# Autodesk Inventor assembly: gun 3_ЗЕРКАЛО1
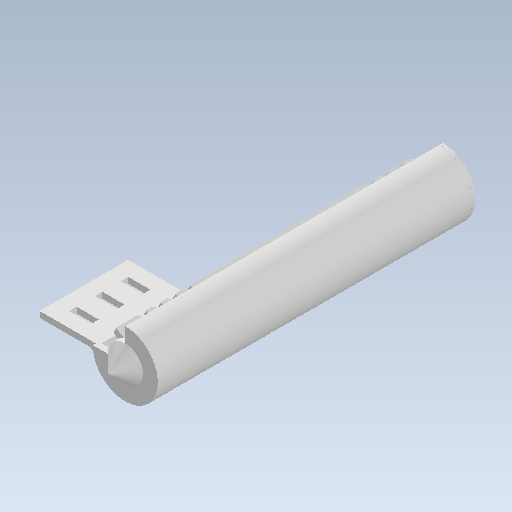
[picture p0: Inventor's stored thumbnail of the model, 512x512]
Saved by Autodesk Inventor 2020.1 (Build 241239000, 239)
## iProperties
Created: 2022-04-02
Part Number: gun 3_ЗЕРКАЛО1
Document SubType Name: Assembly
Designer: User
Author: User
## Documents named in this file (8)
- D:\GitHub\TANK\3D-turret\gun 3_ЗЕРКАЛО1.iam
- D:\GitHub\TANK\3D-turret\barrel_holder_ЗЕРКАЛО1.ipt
- D:\GitHub\TANK\3D-turret\trunk_ЗЕРКАЛО1.ipt
- D:\GitHub\TANK\3D-turret\ось пушки 3_ЗЕРКАЛО1.ipt
- D:\GitHub\TANK\3D-turret\подшипник_ЗЕРКАЛО1.ipt
- D:\GitHub\TANK\3D-turret\кожух пушки_ЗЕРКАЛО1.ipt
- D:\GitHub\TANK\3D-turret\крышка кожуха пушки_ЗЕРКАЛО1.ipt
- D:\GitHub\TANK\3D-turret\крышка кожуха пушки_ЗЕРКАЛО_ЗЕРКАЛО.ipt
## Components (14 placed, 7 different names)
1. barrel_holder_ЗЕРКАЛО1:1 — Жесткий:1, Жесткий:3
2. barrel_holder_ЗЕРКАЛО1:2 — Жесткий:2
3. ось пушки 3_ЗЕРКАЛО1:1 — Жесткий:3, Жесткий:4, Жесткий:5
4. подшипник_ЗЕРКАЛО1:1 — Жесткий:4
5. подшипник_ЗЕРКАЛО1:2 — Совмещение:1, Жесткий:5
6. кожух пушки_ЗЕРКАЛО1:1 — Жесткий:6, Жесткий:7
7. крышка кожуха пушки_ЗЕРКАЛО1:1 — Жесткий:6
8. крышка кожуха пушки_ЗЕРКАЛО_ЗЕРКАЛО:1 — Совмещение:1, Жесткий:7
9. trunk_ЗЕРКАЛО1:1 — Жесткий:1
10. trunk_ЗЕРКАЛО1:2
11. trunk_ЗЕРКАЛО1:3 — Жесткий:2
12. trunk_ЗЕРКАЛО1:4
13. trunk_ЗЕРКАЛО1:5
14. trunk_ЗЕРКАЛО1:6
## Component patterns: (6 elements, first: trunk_ЗЕРКАЛО1:1)
## Relationships (8: WeldJoint 7, Mate 1)
- Совмещение:1 [Mate]: подшипник_ЗЕРКАЛО1:2 ↔ крышка кожуха пушки_ЗЕРКАЛО_ЗЕРКАЛО:1
- Жесткий:1 [WeldJoint]: barrel_holder_ЗЕРКАЛО1:1 ↔ trunk_ЗЕРКАЛО1:1
- Жесткий:3 [WeldJoint]: barrel_holder_ЗЕРКАЛО1:1 ↔ ось пушки 3_ЗЕРКАЛО1:1
- Жесткий:4 [WeldJoint]: ось пушки 3_ЗЕРКАЛО1:1 ↔ подшипник_ЗЕРКАЛО1:1
- Жесткий:5 [WeldJoint]: ось пушки 3_ЗЕРКАЛО1:1 ↔ подшипник_ЗЕРКАЛО1:2
- Жесткий:6 [WeldJoint]: кожух пушки_ЗЕРКАЛО1:1 ↔ крышка кожуха пушки_ЗЕРКАЛО1:1
- Жесткий:7 [WeldJoint]: кожух пушки_ЗЕРКАЛО1:1 ↔ крышка кожуха пушки_ЗЕРКАЛО_ЗЕРКАЛО:1
- Жесткий:2 [WeldJoint]: barrel_holder_ЗЕРКАЛО1:2 ↔ trunk_ЗЕРКАЛО1:3
